# Autodesk Inventor assembly: Entrance Assembly
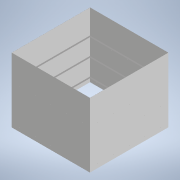
[picture p0: Inventor's stored thumbnail of the model, 180x180]
Saved by Autodesk Inventor 2022 (Build 260153000, 153)
## iProperties
Created: 2022-03-06
Part Number: Entrance Assembly
Document SubType Name: Assembly
Designer: calvi
Author: calvi
## Documents named in this file (3)
- E:\Dr. A Muchiri\Wind tunnel_Dr.A Muchiri\Entrance Assembly.iam
- E:\Dr. A Muchiri\Wind tunnel_Dr.A Muchiri\Entrance.ipt
- E:\Dr. A Muchiri\Wind tunnel_Dr.A Muchiri\HoneyComb Frame.ipt
## Components (4 placed, 2 different names)
1. Entrance:1 — Flush:1, Flush:2, Flush:3, Flush:4, Mate:1, Mate:2, Mate:3, Mate:4, Mate:5, Mate:6, Mate:7, Mate:8, Mate:9, Mate:10, Mate:11
2. HoneyComb Frame:1 — Flush:1, Flush:2, Flush:3, Flush:4, Mate:1, Mate:2, Mate:3, Mate:4, Mate:5
3. HoneyComb Frame:2 — Mate:6, Mate:7, Mate:8
4. HoneyComb Frame:3 — Mate:9, Mate:10, Mate:11
## Relationships (15: Mate 11, Flush 4)
- Flush:1: Entrance:1 ↔ HoneyComb Frame:1
- Flush:2: Entrance:1 ↔ HoneyComb Frame:1
- Flush:3: Entrance:1 ↔ HoneyComb Frame:1
- Flush:4: Entrance:1 ↔ HoneyComb Frame:1
- Mate:1: Entrance:1 ↔ HoneyComb Frame:1
- Mate:2: Entrance:1 ↔ HoneyComb Frame:1
- Mate:3: Entrance:1 ↔ HoneyComb Frame:1
- Mate:4: Entrance:1 ↔ HoneyComb Frame:1
- Mate:5: Entrance:1 ↔ HoneyComb Frame:1
- Mate:6: Entrance:1 ↔ HoneyComb Frame:2
- Mate:7: Entrance:1 ↔ HoneyComb Frame:2
- Mate:8: Entrance:1 ↔ HoneyComb Frame:2
- Mate:9: Entrance:1 ↔ HoneyComb Frame:3
- Mate:10: Entrance:1 ↔ HoneyComb Frame:3
- Mate:11: Entrance:1 ↔ HoneyComb Frame:3
